# Autodesk Inventor assembly: Joint Assembly
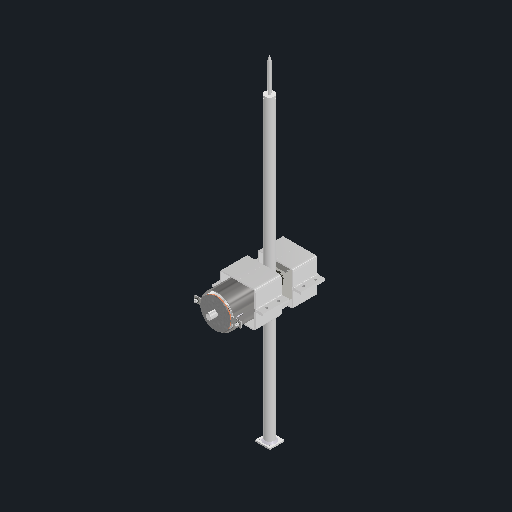
[picture p0: Inventor's stored thumbnail of the model, 512x512]
Saved by Autodesk Inventor 2026.3 (Build 303398000, 398)
## iProperties
Created: 2026-07-22
Part Number: Joint Assembly
Document SubType Name: Assembly
Designer: matot
Author: matot
## Documents named in this file (16)
- C:\Users\matot\OneDrive - Stellenbosch University\2026\MechatronicsProject478\Building the joint\Joint Assembly\Joint Assembly.iam
- C:\Users\matot\OneDrive - Stellenbosch University\2026\MechatronicsProject478\Building the joint\Joint Assembly\Final joint shaft.ipt
- C:\Users\matot\OneDrive - Stellenbosch University\2026\MechatronicsProject478\Building the joint\Joint Assembly\2058786.iam
- C:\Users\matot\OneDrive - Stellenbosch University\2026\MechatronicsProject478\Building the joint\Joint Assembly\8236967.ipt
- C:\Users\matot\OneDrive - Stellenbosch University\2026\MechatronicsProject478\Building the joint\Joint Assembly\Optical Encoder.ipt
- C:\Users\matot\OneDrive - Stellenbosch University\2026\MechatronicsProject478\Building the joint\Joint Assembly\Bearing housing top.ipt
- C:\Users\matot\OneDrive - Stellenbosch University\2026\MechatronicsProject478\Building the joint\Joint Assembly\Bearing housing bottom.ipt
- C:\Users\matot\OneDrive - Stellenbosch University\2026\MechatronicsProject478\Building the joint\Joint Assembly\Joint Housing Bottom_final.iam
- C:\Users\matot\OneDrive - Stellenbosch University\2026\MechatronicsProject478\Building the joint\Joint Assembly\Complete front top housing.iam
- C:\Users\matot\OneDrive - Stellenbosch University\2026\MechatronicsProject478\Building the joint\Joint Assembly\Complete back top housing.iam
- C:\Users\matot\OneDrive - Stellenbosch University\2026\MechatronicsProject478\Building the joint\Joint Assembly\Base link.iam
- C:\Users\matot\OneDrive - Stellenbosch University\2026\MechatronicsProject478\Building the joint\Joint Assembly\Output Link.iam
- C:\Users\matot\OneDrive - Stellenbosch University\2026\MechatronicsProject478\Building the joint\Joint Assembly\Key.ipt
- C:\Users\matot\OneDrive - Stellenbosch University\2026\MechatronicsProject478\Building the joint\Joint Assembly\Electromanetic brake.iam
- C:\Users\matot\OneDrive - Stellenbosch University\2026\MechatronicsProject478\Building the joint\Joint Assembly\Friction Plate.ipt
- C:\Users\matot\OneDrive - Stellenbosch University\2026\MechatronicsProject478\Building the joint\Joint Assembly\Brake disc.ipt
## Components (19 placed, 15 different names)
1. Final joint shaft:1 — Insert:1, Insert:2, Mate:1, Insert:5, Tangent:3, Mate:17, Tangent:4, Mate:24, Mate:25, Flush:19, Insert:23, Insert:24, Insert:25
2. 2058786:1 [sub-assembly] — Insert:2, Insert:4, Insert:17, Insert:20
3. 2058786:2 [sub-assembly] — Insert:1, Insert:3, Insert:18, Insert:19
4. 8236967:1 — Insert:4
5. 8236967:2 — Insert:3
6. Optical Encoder:1 — Mate:1, Insert:5
7. Bearing housing top:1 — Insert:17, Mate:14
8. Bearing housing top:2 — Insert:18, Mate:13
9. Bearing housing bottom:1 — Insert:20, Mate:14, Mate:15
10. Bearing housing bottom:2 — Insert:19, Mate:13, Mate:16
11. Joint Housing Bottom_final:2 [sub-assembly] — Mate:11, Flush:11, Flush:12, Flush:13, Mate:12, Flush:14, Mate:15, Mate:16, Insert:21, Insert:22, Flush:20
12. Complete front top housing:1 [sub-assembly] — Mate:11, Flush:11, Flush:12
13. Complete back top housing:1 [sub-assembly] — Flush:13, Mate:12, Flush:14
14. Base link:1 [sub-assembly] — Insert:21, Insert:22
15. Output Link:1 [sub-assembly] — Tangent:3, Mate:17, Tangent:4
16. Key:1 — Mate:24, Mate:25, Flush:19
17. Electromanetic brake:1 [sub-assembly] — Insert:23, Flush:20
18. Friction Plate:1 — Insert:24
19. Brake disc:1 — Insert:25
## Relationships (32: Insert 14, Mate 10, Flush 6, Tangent 2)
- Insert:1: Final joint shaft:1 ↔ 2058786:2
- Insert:2: Final joint shaft:1 ↔ 2058786:1
- Insert:3: 2058786:2 ↔ 8236967:2
- Insert:4: 2058786:1 ↔ 8236967:1
- Mate:1: Final joint shaft:1 ↔ Optical Encoder:1
- Insert:5: Final joint shaft:1 ↔ Optical Encoder:1
- Insert:17: 2058786:1 ↔ Bearing housing top:1
- Insert:18: 2058786:2 ↔ Bearing housing top:2
- Insert:19: 2058786:2 ↔ Bearing housing bottom:2
- Insert:20: 2058786:1 ↔ Bearing housing bottom:1
- Mate:11: Joint Housing Bottom_final:2 ↔ Complete front top housing:1
- Flush:11: Joint Housing Bottom_final:2 ↔ Complete front top housing:1
- Flush:12: Joint Housing Bottom_final:2 ↔ Complete front top housing:1
- Flush:13: Joint Housing Bottom_final:2 ↔ Complete back top housing:1
- Mate:12: Joint Housing Bottom_final:2 ↔ Complete back top housing:1
- Flush:14: Joint Housing Bottom_final:2 ↔ Complete back top housing:1
- Mate:13: Bearing housing top:2 ↔ Bearing housing bottom:2
- Mate:14: Bearing housing top:1 ↔ Bearing housing bottom:1
- Mate:15: Bearing housing bottom:1 ↔ Joint Housing Bottom_final:2
- Mate:16: Bearing housing bottom:2 ↔ Joint Housing Bottom_final:2
- Insert:21: Joint Housing Bottom_final:2 ↔ Base link:1
- Insert:22: Joint Housing Bottom_final:2 ↔ Base link:1
- Tangent:3: Final joint shaft:1 ↔ Output Link:1
- Mate:17: Final joint shaft:1 ↔ Output Link:1
- Tangent:4: Final joint shaft:1 ↔ Output Link:1
- Mate:24: Final joint shaft:1 ↔ Key:1
- Mate:25: Final joint shaft:1 ↔ Key:1
- Flush:19: Final joint shaft:1 ↔ Key:1
- Insert:23 (-143 mm): Final joint shaft:1 ↔ Electromanetic brake:1
- Flush:20: Joint Housing Bottom_final:2 ↔ Electromanetic brake:1
- Insert:24 (-28.4 mm): Final joint shaft:1 ↔ Friction Plate:1
- Insert:25 (-22.3 mm): Final joint shaft:1 ↔ Brake disc:1
